# Autodesk Inventor assembly: assembly1
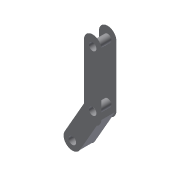
[picture p0: Inventor's stored thumbnail of the model, 180x180]
Saved by Autodesk Inventor 2019 (Build 230136000, 136)
## iProperties
Created: 2019-10-20
Part Number: assembly1
Document SubType Name: Assembly
Designer: DELL PC
Author: DELL PC
## Documents named in this file (3)
- C:\Users\DELL PC\Desktop\Autodesk\assembly1.iam
- C:\Users\DELL PC\Desktop\Autodesk\legfinal.ipt
- C:\Users\DELL PC\Desktop\Autodesk\bel;ow leg.ipt
## Components (2 placed, 2 different names)
1. legfinal:1 — Mate:1, Mate:2
2. bel;ow leg:1 — Mate:1, Mate:2
## Relationships (2: Mate 2)
- Mate:1: legfinal:1 ↔ bel;ow leg:1
- Mate:2: legfinal:1 ↔ bel;ow leg:1
